# Autodesk Inventor assembly: Ring Funnel
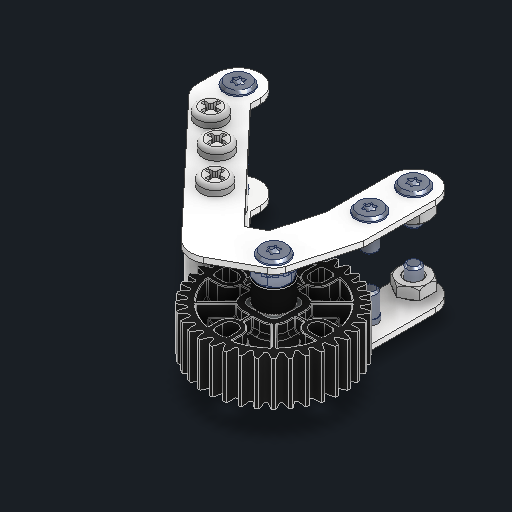
[picture p0: Inventor's stored thumbnail of the model, 512x512]
Saved by Autodesk Inventor 2025.1 (Build 291241000, 241)
## iProperties
Created: 2024-12-17
Part Number: Ring Funnel
Document SubType Name: Assembly
Designer: Averey Ku
Author: Averey Ku
## Documents named in this file (20)
- C:\Users\avere\VEX\High Stakes\CAD\V4\Chassis\Drivebay Left\Ring Funnel.iam
- C:\Users\avere\VEX\High Stakes\CAD\V4\Chassis\Drivebay Left\Custom Parts\Ring Funnel.ipt
- C:\Users\avere\VEX\High Stakes\CAD\ROBOPROS-CAD-Inventor\Motion\Spacers\Spacer Nylon .375 OD\NSpacer .375 OD x .500.ipt
- D:\VEX\High Stakes\CAD\ROBOPROS-CAD-Inventor\Motion\Spacers\Spacer Nylon .375 OD.ipt
- C:\Users\avere\VEX\High Stakes\CAD\ROBOPROS-CAD-Inventor\Motion\Spacers\Spacer Nylon .500 OD\NSpacer White .500 OD x .500.ipt
- D:\VEX\High Stakes\CAD\ROBOPROS-CAD-Inventor\Motion\Spacers\Spacer Nylon .500 OD.ipt
- C:\Users\avere\VEX\High Stakes\CAD\ROBOPROS-CAD-Inventor\Motion\Gears\HS Gear\HS 36T Gear, No Insert.iam
- D:\VEX\High Stakes\CAD\ROBOPROS-CAD-Inventor\Motion\Gears\HS Gear.iam
- C:\Users\avere\VEX\High Stakes\CAD\ROBOPROS-CAD-Inventor\Structure\Hardware\Screw Nylon - Pan Head\NScrew Pan Head Threaded 1.250.ipt
- C:\Users\avere\VEX\High Stakes\CAD\ROBOPROS-CAD-Inventor\Structure\Hardware\Screw Steel - Star\SScrew Star Smooth 1.250.ipt
- D:\VEX\High Stakes\CAD\ROBOPROS-CAD-Inventor\Structure\Hardware\Screw Steel - Star.ipt
- C:\Users\avere\VEX\High Stakes\CAD\ROBOPROS-CAD-Inventor\Structure\Hardware\Nut Nylon Thread-Forming.ipt
- C:\Users\avere\VEX\High Stakes\CAD\ROBOPROS-CAD-Inventor\Structure\Hardware\Screw Shoulder Robosource\SScrew Shoulder Smooth .375 x .12.ipt
- D:\VEX\High Stakes\CAD\ROBOPROS-CAD-Inventor\Structure\Hardware\Screw Shoulder Robosource.ipt
- C:\Users\avere\VEX\High Stakes\CAD\ROBOPROS-CAD-Inventor\Motion\Spacers\Washer Steel\SWasher .375 OD x .062500.ipt
- D:\VEX\High Stakes\CAD\ROBOPROS-CAD-Inventor\Motion\Spacers\Washer Steel.ipt
- C:\Users\avere\VEX\High Stakes\CAD\ROBOPROS-CAD-Inventor\Motion\Spacers\Washer Steel\SWasher .375 OD x .031250.ipt
- C:\Users\avere\VEX\High Stakes\CAD\ROBOPROS-CAD-Inventor\Structure\Hardware\Nut Keps.ipt
- C:\Users\avere\VEX\High Stakes\CAD\ROBOPROS-CAD-Inventor\Motion\Spacers\Spacer Nylon .375 OD\NSpacer .375 OD x .250.ipt
- C:\Users\avere\VEX\High Stakes\CAD\ROBOPROS-CAD-Inventor\Motion\Spacers\Spacer Nylon .375 OD.ipt
## Components (30 placed, 12 different names)
1. Ring Funnel:1 — Insert:23, Insert:27
2. Ring Funnel:2 — Insert:24, Insert:26
3. NSpacer .375 OD x .500:1
4. NSpacer .375 OD x .500:2
5. NSpacer White .500 OD x .500:1
6. NSpacer White .500 OD x .500:2
7. HS 36T Gear, No Insert:1 [sub-assembly]
8. NSpacer White .500 OD x .500:3
9. NSpacer White .500 OD x .500:4
10. NScrew Pan Head Threaded 1.250:1
11. NScrew Pan Head Threaded 1.250:2
12. SScrew Star Smooth 1.250:1
13. NScrew Pan Head Threaded 1.250:3
14. Nut Nylon Thread-Forming:1
15. Nut Nylon Thread-Forming:2
16. Nut Nylon Thread-Forming:3
17. Nut Nylon Thread-Forming:4
18. SScrew Shoulder Smooth .375 x .12:1
19. SScrew Shoulder Smooth .375 x .12:2
20. SScrew Shoulder Smooth .375 x .12:3
21. SScrew Shoulder Smooth .375 x .12:4
22. SScrew Shoulder Smooth .375 x .12:5
23. SScrew Shoulder Smooth .375 x .12:6
24. Nut Nylon Thread-Forming:5 — Insert:23
25. Nut Nylon Thread-Forming:6 — Insert:24
26. SWasher .375 OD x .062500:1 — Insert:25, Insert:26
27. SWasher .375 OD x .031250:2 — Insert:25
28. Nut Keps:1 — Insert:27, Insert:29
29. SWasher .375 OD x .062500:3 — Insert:28
30. NSpacer .375 OD x .250:3 — Insert:28, Insert:29
## Relationships (30: Insert 29, Mate 1)
- [Insert] (25.4 mm): Ring Funnel:1 ↔ Ring Funnel:2
- [Mate]: Ring Funnel:1 ↔ Ring Funnel:2
- [Insert]: NSpacer .375 OD x .500:1 ↔ NSpacer .375 OD x .500:2
- [Insert]: Ring Funnel:1 ↔ NSpacer .375 OD x .500:2
- [Insert]: NSpacer White .500 OD x .500:1 ↔ NSpacer White .500 OD x .500:2
- [Insert]: Ring Funnel:1 ↔ NSpacer White .500 OD x .500:2
- [Insert] (2.3813 mm): Ring Funnel:2 ↔ HS 36T Gear, No Insert:1
- [Insert]: NSpacer White .500 OD x .500:3 ↔ NSpacer White .500 OD x .500:4
- [Insert]: Ring Funnel:2 ↔ NSpacer White .500 OD x .500:3
- [Insert]: Ring Funnel:1 ↔ NScrew Pan Head Threaded 1.250:2
- [Insert]: Ring Funnel:1 ↔ NScrew Pan Head Threaded 1.250:1
- [Insert]: Ring Funnel:1 ↔ SScrew Star Smooth 1.250:1
- [Insert]: Ring Funnel:1 ↔ NScrew Pan Head Threaded 1.250:3
- [Insert]: Ring Funnel:2 ↔ Nut Nylon Thread-Forming:1
- [Insert]: Ring Funnel:2 ↔ Nut Nylon Thread-Forming:2
- [Insert]: Ring Funnel:2 ↔ Nut Nylon Thread-Forming:3
- [Insert]: Ring Funnel:2 ↔ Nut Nylon Thread-Forming:4
- [Insert]: Ring Funnel:1 ↔ SScrew Shoulder Smooth .375 x .12:2
- [Insert]: Ring Funnel:1 ↔ SScrew Shoulder Smooth .375 x .12:3
- [Insert]: Ring Funnel:1 ↔ SScrew Shoulder Smooth .375 x .12:1
- [Insert]: Ring Funnel:2 ↔ SScrew Shoulder Smooth .375 x .12:5
- [Insert]: Ring Funnel:2 ↔ SScrew Shoulder Smooth .375 x .12:4
- [Insert]: Ring Funnel:2 ↔ SScrew Shoulder Smooth .375 x .12:6
- Insert:23 (1.5875 mm): Ring Funnel:1 ↔ Nut Nylon Thread-Forming:5
- Insert:24 (1.5875 mm): Ring Funnel:2 ↔ Nut Nylon Thread-Forming:6
- Insert:25: SWasher .375 OD x .062500:1 ↔ SWasher .375 OD x .031250:2
- Insert:26: Ring Funnel:2 ↔ SWasher .375 OD x .062500:1
- Insert:27: Ring Funnel:1 ↔ Nut Keps:1
- Insert:28: SWasher .375 OD x .062500:3 ↔ NSpacer .375 OD x .250:3
- Insert:29: Nut Keps:1 ↔ NSpacer .375 OD x .250:3
## Named parameters: d26_d23 = 0 mm, d9_d19 = 25.4 mm, d10_d20 = 0 mm, d11_d21 = 0 mm, d12_d22 = 0 mm
